# Autodesk Inventor assembly: outer
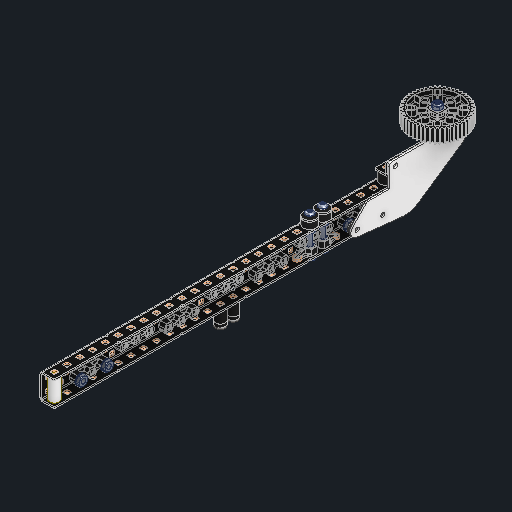
[picture p0: Inventor's stored thumbnail of the model, 512x512]
Saved by Autodesk Inventor 2024 (Build 280153000, 153)
## iProperties
Created: 2024-02-10
Part Number: outer
Document SubType Name: Assembly
Designer: Averey Ku
Author: Averey Ku
## Documents named in this file (19)
- D:\vex_robotics\hardware\cad\vroomba_v0.1\chassis\drivebay\outer.iam
- D:\vex_robotics\hardware\cad\VEX-CAD-Inventor-1.41\Structure\C Channel\Aluminum 1x2x1\Alu C 1x2x1x28.ipt
- D:\vex_robotics\hardware\cad\VEX-CAD-Inventor-1.41\Motion\Shaft LS\Bearing Flat Low Profile.ipt
- D:\vex_robotics\hardware\cad\hardware\.375 OD Aluminum Spacer 0.875.ipt
- D:\vex_robotics\hardware\cad\VEX-CAD-Inventor-1.41\Structure\Hardware\Nut Keps.ipt
- D:\vex_robotics\hardware\cad\VEX-CAD-Inventor-1.41\Motion\Spacers\Spacer Nylon .500 OD\NSpacer Black .500 OD x .250.ipt
- D:\vex_robotics\hardware\cad\VEX-CAD-Inventor-1.41\Motion\Spacers\Spacer Nylon .500 OD.ipt
- D:\vex_robotics\hardware\cad\VEX-CAD-Inventor-1.41\Motion\Spacers\Washer Delrin\DWasher .500 OD x .062500.ipt
- D:\vex_robotics\hardware\cad\VEX-CAD-Inventor-1.41\Structure\Hardware\Nut Hex.ipt
- D:\vex_robotics\hardware\cad\VEX-CAD-Inventor-1.41\Structure\Hardware\Screw Shoulder Robosource.ipt
- D:\vex_robotics\hardware\cad\VEX-CAD-Inventor-1.41\Structure\Hardware\Nut Low Profile.ipt
- D:\vex_robotics\hardware\cad\VEX-CAD-Inventor-1.41\Structure\1-Post Standoff Retainer.ipt
- D:\vex_robotics\hardware\cad\VEX-CAD-Inventor-1.41\Structure\Hardware\Screw Shoulder Robosource\SScrew Shoulder Smooth 1.500 x .18.ipt
- D:\vex_robotics\hardware\cad\vroomba_v0.1\chassis\drivebay\rear_bumper.iam
- D:\vex_robotics\hardware\cad\VEX-CAD-Inventor-1.41\Motion\Spacers\Spacer Nylon .375 OD\NSpacer .375 OD x .500.ipt
- D:\vex_robotics\hardware\cad\VEX-CAD-Inventor-1.41\Motion\Spacers\Spacer Nylon .375 OD.ipt
- D:\vex_robotics\hardware\cad\VEX-CAD-Inventor-1.41\Motion\Spacers\Spacer Nylon .375 OD\NSpacer .375 OD x .125.ipt
- D:\vex_robotics\hardware\cad\VEX-CAD-Inventor-1.41\Motion\Spacers\Washer Steel\SWasher .375 OD x .062500.ipt
- D:\vex_robotics\hardware\cad\VEX-CAD-Inventor-1.41\Motion\Spacers\Washer Steel.ipt
## Components (35 placed, 14 different names)
1. Alu C 1x2x1x28:1 — Insert:1, Mate:1, Insert:2, Mate:2, Insert:3, Mate:3, Insert:4, Mate:4, Insert:5, Mate:5, Insert:6, Mate:6, Insert:7, Mate:7, Insert:8, Insert:9, Insert:14, Insert:15, Insert:20, Mate:8, Insert:21, Mate:9, Insert:24, Insert:25, Insert:28, Insert:29, Insert:34, Mate:10, Insert:37, Insert:40
2. Bearing Flat Low Profile:1 — Insert:1, Mate:1, Insert:30, Insert:31
3. Bearing Flat Low Profile:2 — Insert:2, Mate:2
4. Bearing Flat Low Profile:3 — Insert:3, Mate:3
5. Bearing Flat Low Profile:4 — Insert:4, Mate:4, Insert:32, Insert:33
6. Bearing Flat Low Profile:5 — Insert:5, Mate:5
7. Bearing Flat Low Profile:6 — Insert:6, Mate:6
8. Bearing Flat Low Profile:7 — Insert:7, Mate:7
9. .375 OD Aluminum Spacer 0.875:1 — Insert:8
10. .375 OD Aluminum Spacer 0.875:2 — Insert:9
11. Nut Keps:3 — Insert:14
12. Nut Keps:4 — Insert:15
13. Nut Low Profile:1 — Insert:19
14. Nut Low Profile:2 — Insert:18
15. 1-Post Standoff Retainer:1 — Insert:18, Insert:21, Mate:9
16. 1-Post Standoff Retainer:2 — Insert:19, Insert:20, Mate:8
17. NSpacer Black .500 OD x .250:1 — Insert:23, Insert:25
18. NSpacer Black .500 OD x .250:2 — Insert:22, Insert:24
19. DWasher .500 OD x .062500:1 — Insert:23, Insert:27
20. DWasher .500 OD x .062500:2 — Insert:22, Insert:26
21. SScrew Shoulder Smooth 1.500 x .18:1 — Insert:27
22. SScrew Shoulder Smooth 1.500 x .18:2 — Insert:26
23. Nut Hex:1 — Insert:28
24. Nut Hex:2 — Insert:29
25. Nut Keps:5 — Insert:31
26. Nut Keps:6 — Insert:30
27. Nut Keps:7 — Insert:33
28. Nut Keps:8 — Insert:32
29. rear_bumper:1 [sub-assembly] — Insert:34, Mate:10
30. NSpacer .375 OD x .500:1 — Insert:36, Insert:37
31. NSpacer .375 OD x .125:2 — Insert:35, Insert:36
32. SWasher .375 OD x .062500:1 — Insert:35
33. NSpacer .375 OD x .500:3 — Insert:40
34. NSpacer .375 OD x .125:4
35. SWasher .375 OD x .062500:2
## Relationships (44: Insert 34, Mate 10)
- Insert:1: Alu C 1x2x1x28:1 ↔ Bearing Flat Low Profile:1
- Mate:1: Alu C 1x2x1x28:1 ↔ Bearing Flat Low Profile:1
- Insert:2: Alu C 1x2x1x28:1 ↔ Bearing Flat Low Profile:2
- Mate:2: Alu C 1x2x1x28:1 ↔ Bearing Flat Low Profile:2
- Insert:3: Alu C 1x2x1x28:1 ↔ Bearing Flat Low Profile:3
- Mate:3: Alu C 1x2x1x28:1 ↔ Bearing Flat Low Profile:3
- Insert:4: Alu C 1x2x1x28:1 ↔ Bearing Flat Low Profile:4
- Mate:4: Alu C 1x2x1x28:1 ↔ Bearing Flat Low Profile:4
- Insert:5: Alu C 1x2x1x28:1 ↔ Bearing Flat Low Profile:5
- Mate:5: Alu C 1x2x1x28:1 ↔ Bearing Flat Low Profile:5
- Insert:6: Alu C 1x2x1x28:1 ↔ Bearing Flat Low Profile:6
- Mate:6: Alu C 1x2x1x28:1 ↔ Bearing Flat Low Profile:6
- Insert:7: Alu C 1x2x1x28:1 ↔ Bearing Flat Low Profile:7
- Mate:7: Alu C 1x2x1x28:1 ↔ Bearing Flat Low Profile:7
- Insert:8: Alu C 1x2x1x28:1 ↔ .375 OD Aluminum Spacer 0.875:1
- Insert:9: Alu C 1x2x1x28:1 ↔ .375 OD Aluminum Spacer 0.875:2
- Insert:14: Alu C 1x2x1x28:1 ↔ Nut Keps:3
- Insert:15: Alu C 1x2x1x28:1 ↔ Nut Keps:4
- Insert:18: Nut Low Profile:2 ↔ 1-Post Standoff Retainer:1
- Insert:19: Nut Low Profile:1 ↔ 1-Post Standoff Retainer:2
- Insert:20: Alu C 1x2x1x28:1 ↔ 1-Post Standoff Retainer:2
- Mate:8: Alu C 1x2x1x28:1 ↔ 1-Post Standoff Retainer:2
- Insert:21: Alu C 1x2x1x28:1 ↔ 1-Post Standoff Retainer:1
- Mate:9: Alu C 1x2x1x28:1 ↔ 1-Post Standoff Retainer:1
- Insert:22: NSpacer Black .500 OD x .250:2 ↔ DWasher .500 OD x .062500:2
- Insert:23: NSpacer Black .500 OD x .250:1 ↔ DWasher .500 OD x .062500:1
- Insert:24: Alu C 1x2x1x28:1 ↔ NSpacer Black .500 OD x .250:2
- Insert:25: Alu C 1x2x1x28:1 ↔ NSpacer Black .500 OD x .250:1
- Insert:26 (1.5875 mm): DWasher .500 OD x .062500:2 ↔ SScrew Shoulder Smooth 1.500 x .18:2
- Insert:27 (1.5875 mm): DWasher .500 OD x .062500:1 ↔ SScrew Shoulder Smooth 1.500 x .18:1
- Insert:28: Alu C 1x2x1x28:1 ↔ Nut Hex:1
- Insert:29: Alu C 1x2x1x28:1 ↔ Nut Hex:2
- Insert:30 (1.27 mm): Bearing Flat Low Profile:1 ↔ Nut Keps:6
- Insert:31 (1.27 mm): Bearing Flat Low Profile:1 ↔ Nut Keps:5
- Insert:32 (1.27 mm): Bearing Flat Low Profile:4 ↔ Nut Keps:8
- Insert:33 (1.27 mm): Bearing Flat Low Profile:4 ↔ Nut Keps:7
- Insert:34: Alu C 1x2x1x28:1 ↔ rear_bumper:1
- Mate:10: Alu C 1x2x1x28:1 ↔ rear_bumper:1
- Insert:35: NSpacer .375 OD x .125:2 ↔ SWasher .375 OD x .062500:1
- Insert:36: NSpacer .375 OD x .500:1 ↔ NSpacer .375 OD x .125:2
- Insert:37: Alu C 1x2x1x28:1 ↔ NSpacer .375 OD x .500:1
- [Insert]: NSpacer .375 OD x .125:4 ↔ SWasher .375 OD x .062500:2
- [Insert]: NSpacer .375 OD x .500:3 ↔ NSpacer .375 OD x .125:4
- Insert:40: Alu C 1x2x1x28:1 ↔ NSpacer .375 OD x .500:3
## Named parameters: d58_d55 = 0 mm, d59_d56 = 0 mm
